# Autodesk Inventor assembly: ASY 000 ДМФ Disk Micro filter v3.0
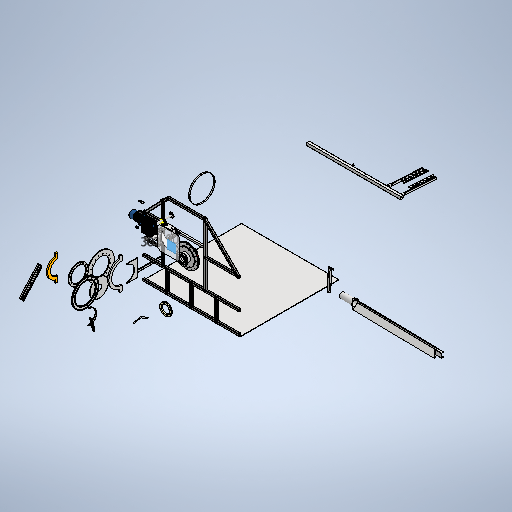
[picture p0: Inventor's stored thumbnail of the model, 512x512]
Saved by Autodesk Inventor 2026.2 (Build 302298010, 298A)
## iProperties
Part Number: ASY 000 ДМФ Disk Micro filter v3.0
Document SubType Name: Assembly
Designer: admin
Author: admin
## Documents named in this file (46)
- C:\Users\admin\Documents\Inventor\DMF-Disk-Micro-Filter\ASY 000 ДМФ Disk Micro filter v3.0.iam
- C:\Users\admin\Documents\Inventor\DMF-Disk-Micro-Filter\Wall right v2.0.ipt
- C:\Users\admin\Documents\Inventor\DMF-Disk-Micro-Filter\DF1.03 Wall bottom v2.0.ipt
- C:\Users\admin\Documents\Inventor\DMF-Disk-Micro-Filter\DF1.04 Wall face v2.0.ipt
- C:\Users\admin\Documents\Inventor\DMF-Disk-Micro-Filter\ДМФ 021 кольцо прижимное нос v2.0.ipt
- C:\Users\admin\Documents\Inventor\DMF-Disk-Micro-Filter\ДМФ 032 крышка Нос v2.0.ipt
- C:\Users\admin\Documents\Inventor\DMF-Disk-Micro-Filter\ДМФ 091 Постель НОС v2.0.ipt
- C:\Users\admin\Documents\Inventor\DMF-Disk-Micro-Filter\ДМФ 022 кольцо прижимное корма v2.0.ipt
- C:\Users\admin\Documents\Inventor\DMF-Disk-Micro-Filter\ДМФ 093 Постель КОРМА v2.0.ipt
- C:\Users\admin\Documents\Inventor\DMF-Disk-Micro-Filter\ДМФ 092 Коромысло КОРМА v2.0.ipt
- C:\Users\admin\Documents\Inventor\DMF-Disk-Micro-Filter\ДМФ 055 труба илоотвода v2.0.ipt
- C:\Users\admin\Documents\Inventor\DMF-Disk-Micro-Filter\ДМФ 033 держатель лотка v2.0.ipt
- C:\Users\admin\Documents\Inventor\DMF-Disk-Micro-Filter\ASY ДМФ лоток 050 илоотвод v2.0.iam
- C:\Users\admin\Documents\Inventor\DMF-Disk-Micro-Filter\ДМФ 092 Коромысло НОС v2.0.ipt
- C:\Users\admin\Documents\Inventor\DMF-Disk-Micro-Filter\ДМФ 066 Гребенка v2.0.ipt
- C:\Users\admin\Documents\Inventor\DMF-Disk-Micro-Filter\ДМФ 025 кольцо прижимное корма наружное v2.0.ipt
- C:\Users\admin\Documents\Inventor\DMF-Disk-Micro-Filter\ДМФ 067 крышка v2.0.ipt
- C:\Users\admin\Documents\Inventor\DMF-Disk-Micro-Filter\ДМФ 081 труба форсунки v2.0.ipt
- C:\Users\admin\Documents\Inventor\DMF-Disk-Micro-Filter\ASY Обрешетка лицевая стенка.iam
- C:\Users\admin\Documents\Inventor\DMF-Disk-Micro-Filter\Вал ведущей шестерни.ipt
- C:\Users\admin\Documents\Inventor\DMF-Disk-Micro-Filter\Корпусный подшипник D35.ipt
- C:\Users\admin\Documents\Inventor\DMF-Disk-Micro-Filter\Мотор-редуктор NMRV 090(80B5).ipt
- C:\Users\admin\Documents\Inventor\DMF-Disk-Micro-Filter\DMF pancake.ipt
- C:\Users\admin\Documents\Inventor\DMF-Disk-Micro-Filter\Нога для постели.ipt
- C:\Users\admin\Documents\Inventor\DMF-Disk-Micro-Filter\Нога для постели №2.ipt
- C:\Users\admin\Documents\Inventor\DMF-Disk-Micro-Filter\ДМФ 092 Постель НОС v2.0.ipt
- C:\Users\admin\Documents\Inventor\DMF-Disk-Micro-Filter\ДМФ 094 Постель НОС крепление v2.0.ipt
- C:\Users\admin\Documents\Inventor\DMF-Disk-Micro-Filter\DMF Hat 2.0.ipt
- C:\Users\admin\Documents\Inventor\DMF-Disk-Micro-Filter\DMF Flange exit 2.0.ipt
- C:\Users\admin\Documents\Inventor\DMF-Disk-Micro-Filter\Барабан v2.1\ASY ДМФ 0100 Барабан v2.1.iam
- C:\Users\admin\Documents\Inventor\DMF-Disk-Micro-Filter\Барабан v2.1\DMF flange small gear.ipt
- C:\Users\admin\Documents\Inventor\DMF-Disk-Micro-Filter\Барабан v2.1\DMF small gear.ipt
- C:\Users\admin\Documents\Inventor\DMF-Disk-Micro-Filter\DMF Support ring tail.ipt
- C:\Users\admin\Documents\Inventor\DMF-Disk-Micro-Filter\DMF 082 коллектор болванка.ipt
- C:\Users\admin\Documents\Inventor\DMF-Disk-Micro-Filter\Барабан v2.1\DMF 2.1 Пластина паза маленькая.ipt
- C:\Users\admin\Documents\Inventor\DMF-Disk-Micro-Filter\Барабан v2.1\DMF 01 12 Барабан усилитель v2.1.ipt
- C:\Users\admin\Documents\Inventor\DMF-Disk-Micro-Filter\Барабан v2.1\DMF 2.1 01 45 Gear ring 5.ipt
- C:\Users\admin\Documents\Inventor\DMF-Disk-Micro-Filter\Барабан v2.1\DMF 2.1 01 46 Gear axis wheel 6.ipt
- C:\Users\admin\Documents\Inventor\DMF-Disk-Micro-Filter\Барабан v2.1\DMF 01 13 Барабан усилитель v2.1.ipt
- C:\Users\admin\Documents\Inventor\DMF-Disk-Micro-Filter\ДМФ 01 12 Барабан усилитель.ipt
- C:\Users\admin\Documents\Inventor\DMF-Disk-Micro-Filter\ДМФ 01 15 Барабан усилитель борта.ipt
- C:\Users\admin\Documents\Inventor\DMF-Disk-Micro-Filter\ДМФ 01 15 Барабан усилитель борта_CPY.ipt
- C:\Users\admin\Documents\Inventor\DMF-Disk-Micro-Filter\Барабан v2.1\DMF flange small gear 2.ipt
- C:\Users\admin\Documents\Inventor\DMF-Disk-Micro-Filter\Left wall v2.0.ipt
- C:\Users\admin\Documents\Inventor\DMF-Disk-Micro-Filter\Барабан v2.1\DMF 01 31 Барабан Опорное кольцо НОС v2.1.ipt
- C:\Users\admin\Documents\Inventor\DMF-Disk-Micro-Filter\Подставка под мотор.iam
## Components (47 placed, 45 different names)
1. Wall right v2.0:1 — Rigid:8, Mate:14
2. DF1.03 Wall bottom v2.0:1 — Mate:10, Mate:11, Rigid:8, Mate:12, Rigid:9, Mate:16
3. DF1.04 Wall face v2.0:1
4. DMF 2.1 01 45 Gear ring 5:1 — Rigid:10, Rigid:11
5. ДМФ 021 кольцо прижимное нос v2.0:1
6. ДМФ 032 крышка Нос v2.0:1
7. ДМФ 091 Постель НОС v2.0:1
8. ДМФ 022 кольцо прижимное корма v2.0:1
9. ДМФ 093 Постель КОРМА v2.0:1 — Rigid:11
10. Постель 204 корма:1
11. ДМФ 055 труба илоотвода v2.0:1
12. ДМФ 033 держатель лотка v2.0:1
13. ASY ДМФ лоток 050 илоотвод v2.0:1 [sub-assembly]
14. ДМФ 092 Коромысло НОС v2.0:1
15. ДМФ 066 Гребенка v2.0:1 — Mate:15, Flush:8, Mate:16
16. ДМФ 025 кольцо прижимное корма наружное v2.0:1
17. ДМФ 067 крышка v2.0:1 — Mate:14, Flush:7
18. ДМФ 081 труба форсунки v2.0:1
19. ASY Обрешетка лицевая стенка:1 [sub-assembly] — Mate:13, Flush:5, Flush:6
20. Вал ведущей шестерни:1 — Rotational:5
21. Корпусный подшипник D35:1 — Angle:1, Mate:19
22. Мотор-редуктор NMRV 090(80B5):1 — Rotational:5, Angle:1
23. DMF pancake:1 — Rotational:6
24. Нога для постели:1
25. Нога для постели №2:1 — Mate:18, Flush:9
26. ДМФ 092 Постель НОС v2.0:1
27. ДМФ 094 Постель НОС крепление v2.0:1
28. DMF Hat 2.0:1
29. DMF Flange exit 2.0:1
30. ASY ДМФ 0100 Барабан v2.1:1 [sub-assembly]
31. flange small gear:1
32. DMF small gear:1 — Rotational:4
33. DMF Support ring tail:1
34. DMF 082 коллектор болванка:1
35. ДМФ 081 труба форсунки v2.0:2
36. DMF 2.1 Пластина паза маленькая:1
37. DMF 01 12 Барабан усилитель v2.1:1
38. DMF 2.1 01 46 Gear axis wheel 6:1
39. ДМФ 01 13 Барабан усилитель v2.0:1
40. ДМФ 01 12 Барабан усилитель:1
41. ДМФ 01 15 Барабан усилитель борта:1
42. ДМФ 01 15 Барабан усилитель борта_CPY:1
43. DMF flange small gear 2:1
44. Left wall v2.0:1 — Rigid:9, Mate:13, Flush:5, Flush:6, Flush:7, Mate:15, Flush:8, Rotational:4, Rotational:6, Rigid:10
45. DMF 01 31 Барабан Опорное кольцо НОС v2.1:1
46. ДМФ 094 Постель НОС крепление v2.0:2
47. Подставка под мотор:1 [sub-assembly] — Mate:18, Mate:19, Flush:9
## Relationships (38: Mate 12, WeldJoint 11, Flush 7, RevoluteJoint 6, CylindricalJoint 1, Angle 1)
- [WeldJoint]: ДМФ 055 труба илоотвода v2.0:1 ↔ DMF Flange exit 2.0:1
- [WeldJoint]: DMF pancake:1 ↔ DMF Hat 2.0:1
- [CylindricalJoint]: ДМФ 055 труба илоотвода v2.0:1 ↔ DMF Hat 2.0:1
- [WeldJoint]: Wall right v2.0:1 ↔ DMF Support ring tail:1
- [RevoluteJoint]: ASY ДМФ 0100 Барабан v2.1:1 ↔ DMF Support ring tail:1
- [RevoluteJoint]: ASY ДМФ 0100 Барабан v2.1:1 ↔ DMF Support ring tail:1
- [WeldJoint]: ДМФ 081 труба форсунки v2.0:1 ↔ DMF 082 коллектор болванка:1
- [WeldJoint]: DMF 082 коллектор болванка:1 ↔ ДМФ 081 труба форсунки v2.0:2
- [Mate]: DMF 082 коллектор болванка:1 ↔ ДМФ 01 15 Барабан усилитель борта:1
- [Mate]: DMF 082 коллектор болванка:1 ↔ ДМФ 01 15 Барабан усилитель борта:1
- [Flush]: ДМФ 033 держатель лотка v2.0:1 ↔ ДМФ 01 15 Барабан усилитель борта_CPY:1
- [RevoluteJoint]: Вал ведущей шестерни:1 ↔ DMF small gear:1
- [WeldJoint]: flange small gear:1 ↔ DMF flange small gear 2:1
- [WeldJoint] (-25 mm): Вал ведущей шестерни:1 ↔ flange small gear:1
- [Flush]: ASY Обрешетка лицевая стенка:1 ↔ Нога для постели №2:1
- [Mate]: ASY Обрешетка лицевая стенка:1 ↔ Нога для постели №2:1
- Mate:10: DF1.03 Wall bottom v2.0:1
- Mate:11: DF1.03 Wall bottom v2.0:1
- Rigid:8 [WeldJoint] (-25 mm): Wall right v2.0:1 ↔ DF1.03 Wall bottom v2.0:1
- Mate:12: DF1.03 Wall bottom v2.0:1
- Rigid:9 [WeldJoint] (-25 mm): DF1.03 Wall bottom v2.0:1 ↔ Left wall v2.0:1
- Mate:13: ASY Обрешетка лицевая стенка:1 ↔ Left wall v2.0:1
- Flush:5: ASY Обрешетка лицевая стенка:1 ↔ Left wall v2.0:1
- Flush:6: ASY Обрешетка лицевая стенка:1 ↔ Left wall v2.0:1
- Mate:14: Wall right v2.0:1 ↔ ДМФ 067 крышка v2.0:1
- Flush:7: ДМФ 067 крышка v2.0:1 ↔ Left wall v2.0:1
- Mate:15: ДМФ 066 Гребенка v2.0:1 ↔ Left wall v2.0:1
- Flush:8 (200 mm): ДМФ 066 Гребенка v2.0:1 ↔ Left wall v2.0:1
- Mate:16: DF1.03 Wall bottom v2.0:1 ↔ ДМФ 066 Гребенка v2.0:1
- Rotational:4 [RevoluteJoint] (-33 mm): DMF small gear:1 ↔ Left wall v2.0:1
- Rotational:5 [RevoluteJoint] (3 mm): Вал ведущей шестерни:1 ↔ Мотор-редуктор NMRV 090(80B5):1
- Rotational:6 [RevoluteJoint]: DMF pancake:1 ↔ Left wall v2.0:1
- Rigid:10 [WeldJoint]: DMF 2.1 01 45 Gear ring 5:1 ↔ Left wall v2.0:1
- Rigid:11 [WeldJoint]: DMF 2.1 01 45 Gear ring 5:1 ↔ ДМФ 093 Постель КОРМА v2.0:1
- Angle:1 (0 deg): Корпусный подшипник D35:1 ↔ Мотор-редуктор NMRV 090(80B5):1
- Mate:18: Нога для постели №2:1 ↔ Подставка под мотор:1
- Mate:19: Корпусный подшипник D35:1 ↔ Подставка под мотор:1
- Flush:9: Нога для постели №2:1 ↔ Подставка под мотор:1
